# Autodesk Inventor assembly: holders
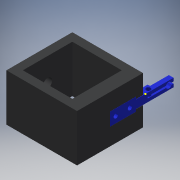
[picture p0: Inventor's stored thumbnail of the model, 180x180]
Saved by Autodesk Inventor 2017 (Build 210142000, 142)
## iProperties
Created: 2018-04-15
Part Number: holders
Document SubType Name: Assembly
Designer: dasae
Author: dasae
## Documents named in this file (3)
- C:\Users\dasae\Documents\Work\Hiwi Neuroelectronic systems\CAD\heatsink\holders.iam
- C:\Users\dasae\Documents\Work\Hiwi Neuroelectronic systems\CAD\heatsink\holder.ipt
- C:\Users\dasae\Documents\Work\Hiwi Neuroelectronic systems\CAD\heatsink\ferrule holder.ipt
## Components (2 placed, 2 different names)
1. holder:1 — Insert:1, Mate:1
2. ferrule holder:1 — Insert:1, Mate:1
## Relationships (2: Insert 1, Mate 1)
- Insert:1: holder:1 ↔ ferrule holder:1
- Mate:1: holder:1 ↔ ferrule holder:1
